# Autodesk Inventor assembly: wheel_raised
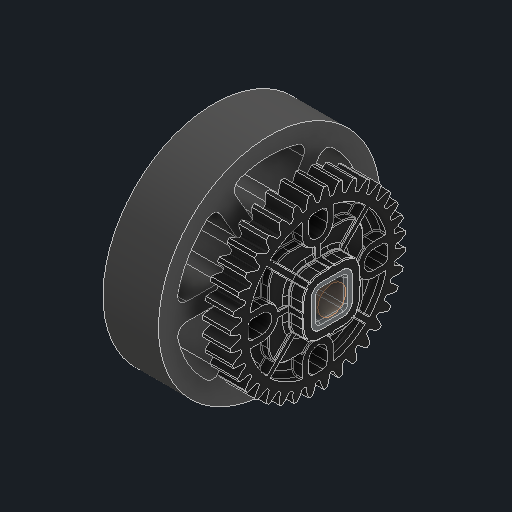
[picture p0: Inventor's stored thumbnail of the model, 512x512]
Saved by Autodesk Inventor 2024 (Build 280153000, 153)
## iProperties
Created: 2024-03-23
Part Number: wheel_raised
Document SubType Name: Assembly
Designer: Averey Ku
Author: Averey Ku
## Documents named in this file (9)
- D:\vex_robotics\hardware\cad\infection\chassis\drivebay\wheel_raised.iam
- D:\vex_robotics\hardware\cad\VEX-CAD-Inventor-1.41\Structure\Hardware\Nut Keps.ipt
- D:\vex_robotics\hardware\cad\VEX-CAD-Inventor-1.41\Motion\Spacers\Washer Steel\SWasher .375 OD x .062500.ipt
- D:\vex_robotics\hardware\cad\VEX-CAD-Inventor-1.41\Motion\Spacers\Washer Steel.ipt
- D:\vex_robotics\hardware\cad\VEX-CAD-Inventor-1.41\Motion\Spacers\Washer Teflon.ipt
- D:\vex_robotics\hardware\cad\VEX-CAD-Inventor-1.41\Motion\Spacers\Washer Teflon\TWasher .375 OD x .03125.ipt
- D:\vex_robotics\hardware\cad\VEX-CAD-Inventor-1.41\Motion\Wheels\Flex Wheels\2.000 Flex Wheel\2.000 60A .500.ipt
- D:\vex_robotics\hardware\cad\VEX-CAD-Inventor-1.41\Motion\Wheels\Flex Wheels\2.000 Flex Wheel.ipt
- D:\vex_robotics\hardware\cad\infection\custom_parts\chassis\drivebay\half_cut_36t.ipt
## Components (5 placed, 5 different names)
1. Nut Keps:1 — Insert:3
2. SWasher .375 OD x .062500:1 — Insert:3, Insert:4
3. TWasher .375 OD x .03125:1 — Insert:4, Insert:5
4. 2.000 60A .500:1 — Insert:5, Insert:6
5. half_cut_36t:1 — Insert:6
## Relationships (4: Insert 4)
- Insert:3: Nut Keps:1 ↔ SWasher .375 OD x .062500:1
- Insert:4: SWasher .375 OD x .062500:1 ↔ TWasher .375 OD x .03125:1
- Insert:5 (1.5875 mm): TWasher .375 OD x .03125:1 ↔ 2.000 60A .500:1
- Insert:6 (1.5875 mm): 2.000 60A .500:1 ↔ half_cut_36t:1
